# Autodesk Inventor assembly: BipeD
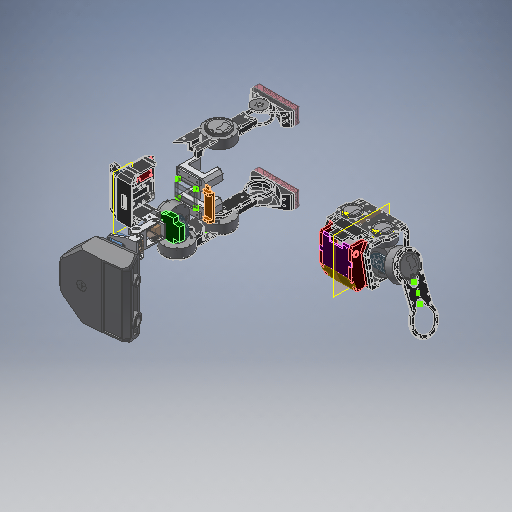
[picture p0: Inventor's stored thumbnail of the model, 512x512]
Saved by Autodesk Inventor 2026 (Build 300175000, 175)
## iProperties
Company: UNSPECIFIED
Created: 1900-01-01
Part Number: BipeD
Description: STEP AP242
Document SubType Name: Assembly
Designer: kirpe
Mass: 5721.04 g
Surface Area: 15487 cm^2
Volume: 5721.04 cm^3
Density: 1 g/cm^3
Sending System: C3D Toolkit
Preprocessor: C3D Converter
Title: Òèíêåð
Author: UNSPECIFIED
Revision Number: ANYUNSPECIFIED
## Documents named in this file (90)
- C:\BE2R\Legged_bot\biped_model\BipeD.iam
- C:\BE2R\Legged_bot\biped_model\Заднее_Ребро.ipt
- C:\BE2R\Legged_bot\biped_model\Переднее_Ребро.ipt
- C:\BE2R\Legged_bot\biped_model\Днище_Корпуса.ipt
- C:\BE2R\Legged_bot\biped_model\Булка.ipt
- C:\BE2R\Legged_bot\biped_model\Булка_1.ipt
- C:\BE2R\Legged_bot\biped_model\Держатель_ТазаV2.ipt
- C:\BE2R\Legged_bot\biped_model\DM_8006.ipt
- C:\BE2R\Legged_bot\biped_model\DM_8006_1.ipt
- C:\BE2R\Legged_bot\biped_model\Держатель_ТазаV2_1.ipt
- C:\BE2R\Legged_bot\biped_model\Тазовая_Прокладка.ipt
- C:\BE2R\Legged_bot\biped_model\БедроV2.ipt
- C:\BE2R\Legged_bot\biped_model\Голень.ipt
- C:\BE2R\Legged_bot\biped_model\Наполнитель_Бедра2.ipt
- C:\BE2R\Legged_bot\biped_model\Наполнитель Голени.ipt
- C:\BE2R\Legged_bot\biped_model\Прокладка_Стопы.ipt
- C:\BE2R\Legged_bot\biped_model\БедроV2_1.ipt
- C:\BE2R\Legged_bot\biped_model\Наполнитель_Бедра2_1.ipt
- C:\BE2R\Legged_bot\biped_model\Наполнитель Голени_1.ipt
- C:\BE2R\Legged_bot\biped_model\Голень_1.ipt
- C:\BE2R\Legged_bot\biped_model\Прокладка_Стопы_1.ipt
- C:\BE2R\Legged_bot\biped_model\НагрудникV2.ipt
- C:\BE2R\Legged_bot\biped_model\Расширитель_РюкзакаV2.ipt
- C:\BE2R\Legged_bot\biped_model\Плата.ipt
- C:\BE2R\Legged_bot\biped_model\Расширитель_РюкзакаV2_1.ipt
- C:\BE2R\Legged_bot\biped_model\СтопаV3.ipt
- C:\BE2R\Legged_bot\biped_model\СтопаV3_1.ipt
- C:\BE2R\Legged_bot\biped_model\Голова.ipt
- C:\BE2R\Legged_bot\biped_model\Шея_Верх.ipt
- C:\BE2R\Legged_bot\biped_model\Шея_Низ.ipt
- C:\BE2R\Legged_bot\biped_model\Крышка_Корпуса.ipt
- C:\BE2R\Legged_bot\biped_model\Крышка_Тумблера.ipt
- C:\BE2R\Legged_bot\biped_model\Стул.ipt
- C:\BE2R\Legged_bot\biped_model\Тумблер.ipt
- C:\BE2R\Legged_bot\biped_model\Качалка_SCS125.ipt
- C:\BE2R\Legged_bot\biped_model\Feetech_SERVO_SCS125.ipt
- C:\BE2R\Legged_bot\biped_model\FeeTech_SCS40.ipt
- C:\BE2R\Legged_bot\biped_model\Тазовая_Прокладка_1.ipt
- C:\BE2R\Legged_bot\biped_model\Кость_Таза.ipt
- C:\BE2R\Legged_bot\biped_model\Кость_Таза_1.ipt
- C:\BE2R\Legged_bot\biped_model\Кассета1.ipt
- C:\BE2R\Legged_bot\biped_model\Кассета2.ipt
- C:\BE2R\Legged_bot\biped_model\Рамка_Рюкзака.ipt
- C:\BE2R\Legged_bot\biped_model\Винт с цилиндрической головкой и шестигранным углублением под ключ ГОСТ Р ИСО 4762 -М3 x 10.ipt
- C:\BE2R\Legged_bot\biped_model\Винт с цилиндрической головкой и шестигранным углублением под ключ ГОСТ Р ИСО 4762-М3 x 6.ipt
- C:\BE2R\Legged_bot\biped_model\Винт с цилиндрической головкой и шестигранным углублением под ключ ГОСТ Р ИСО 4762-М3 x 12.ipt
- C:\BE2R\Legged_bot\biped_model\Винт с цилиндрической головкой и шестигранным углублением под ключ ГОСТ Р ИСО 4762 -М4 x 8.ipt
- C:\BE2R\Legged_bot\biped_model\Винт с цилиндрической головкой и шестигранным углублением под ключ ГОСТ Р ИСО 4762 -М3 x 16.ipt
- C:\BE2R\Legged_bot\biped_model\Винт с цилиндрической головкой и шестигранным углублением под ключ ГОСТ Р ИСО 4762 -М4 x 10.ipt
- C:\BE2R\Legged_bot\biped_model\Винт с цилиндрической головкой и шестигранным углублением под ключ ГОСТ Р ИСО 4762 -М3 x 10_1.ipt
- C:\BE2R\Legged_bot\biped_model\Винт с цилиндрической головкой и шестигранным углублением под ключ ГОСТ Р ИСО 4762-М3 x 6_1.ipt
- C:\BE2R\Legged_bot\biped_model\Винт с цилиндрической головкой и шестигранным углублением под ключ ГОСТ Р ИСО 4762-М3 x 12_1.ipt
- C:\BE2R\Legged_bot\biped_model\Винт с цилиндрической головкой и шестигранным углублением под ключ ГОСТ Р ИСО 4762 -М3 x 16_1.ipt
- C:\BE2R\Legged_bot\biped_model\Винт с цилиндрической головкой и шестигранным углублением под ключ ГОСТ Р ИСО 4762 -М4 x 10_1.ipt
- C:\BE2R\Legged_bot\biped_model\Винт с цилиндрической головкой и шестигранным углублением под ключ ГОСТ Р ИСО 4762 -М4 x 8_1.ipt
- C:\BE2R\Legged_bot\biped_model\Винт с плоской головкой ГОСТ Р ИСО 1580 -М3 x 8.ipt
- C:\BE2R\Legged_bot\biped_model\Винт с плоской головкой ГОСТ Р ИСО 1580 -М3 x 8_1.ipt
- C:\BE2R\Legged_bot\biped_model\Скамейка.ipt
- C:\BE2R\Legged_bot\biped_model\Гайка М3-6H.NF ГОСТ Р 50273-92.ipt
- C:\BE2R\Legged_bot\biped_model\Гайка М3-6H.NF ГОСТ Р 50273-92_1.ipt
- C:\BE2R\Legged_bot\biped_model\Винт с цилиндрической головкой и шестигранным углублением под ключ ГОСТ Р ИСО 4762 -М5 x 16.ipt
- C:\BE2R\Legged_bot\biped_model\Винт с цилиндрической головкой и шестигранным углублением под ключ ГОСТ Р ИСО 4762 -М5 x 16_1.ipt
- C:\BE2R\Legged_bot\biped_model\Гайка М3-6H.NF ГОСТ Р 50273-92_2.ipt
- C:\BE2R\Legged_bot\biped_model\Гайка М3-6H.NF ГОСТ Р 50273-92_3.ipt
- C:\BE2R\Legged_bot\biped_model\Винт с цилиндрической головкой и шестигранным углублением под ключ ГОСТ Р ИСО 4762 -М3 x 20.ipt
- C:\BE2R\Legged_bot\biped_model\Винт с цилиндрической головкой и шестигранным углублением под ключ ГОСТ Р ИСО 4762 -М4 x 20.ipt
- C:\BE2R\Legged_bot\biped_model\Гайка М4-6H.NF ГОСТ Р 50273-92.ipt
- C:\BE2R\Legged_bot\biped_model\Винт с цилиндрической головкой и шестигранным углублением под ключ ГОСТ Р ИСО 4762 -М4 x 12.ipt
- C:\BE2R\Legged_bot\biped_model\Винт с цилиндрической головкой и шестигранным углублением под ключ ГОСТ Р ИСО 4762 -М4 x 16.ipt
- C:\BE2R\Legged_bot\biped_model\Винт с цилиндрической головкой и шестигранным углублением под ключ ГОСТ Р ИСО 4762 -М3 x 20_1.ipt
- C:\BE2R\Legged_bot\biped_model\Винт с плоской головкой ГОСТ Р ИСО 1580 -М3 x 6.ipt
- C:\BE2R\Legged_bot\biped_model\Винт с цилиндрической головкой и шестигранным углублением под ключ ГОСТ Р ИСО 4762 -М3 x 5.ipt
- C:\BE2R\Legged_bot\biped_model\Винт с цилиндрической головкой и шестигранным углублением под ключ ГОСТ Р ИСО 4762-М2,5 x 12.ipt
- C:\BE2R\Legged_bot\biped_model\Гайка М2,5-6H ГОСТ 5916-70.ipt
- C:\BE2R\Legged_bot\biped_model\Тинкер.ipt
- C:\BE2R\Legged_bot\biped_model\Крышка_Платы_Питания.ipt
- C:\BE2R\Legged_bot\biped_model\Переднее_Ребро_1.ipt
- C:\BE2R\Legged_bot\biped_model\Нагрудник_Сторона.ipt
- C:\BE2R\Legged_bot\biped_model\Нагрудник_Сторона_1.ipt
- C:\BE2R\Legged_bot\biped_model\Нагрудник_Низ.ipt
- C:\BE2R\Legged_bot\biped_model\Нагрудник_Середина.ipt
- C:\BE2R\Legged_bot\biped_model\Нагрудник_Центр.ipt
- C:\BE2R\Legged_bot\biped_model\Рюкзак.ipt
- C:\BE2R\Legged_bot\biped_model\Крышка_Рюкзака.ipt
- C:\BE2R\Legged_bot\biped_model\Подставка_Платы.ipt
- C:\BE2R\Legged_bot\biped_model\NONE.ipt
- C:\BE2R\Legged_bot\biped_model\Башмак.ipt
- C:\BE2R\Legged_bot\biped_model\Башмак_1.ipt
- C:\BE2R\Legged_bot\biped_model\Датчик.ipt
- C:\BE2R\Legged_bot\biped_model\DM-J6006.ipt
## Components (355 placed, 86 different names)
1. Заднее_Ребро — Совмещение:10, Совмещение:11, Совмещение:12, Совмещение:41, Совмещение:42
2. Заднее_Ребро:1 — Совмещение:1, Совмещение:2, Совмещение:3, Совмещение:43
3. Переднее_Ребро — Совмещение:4, Совмещение:5, Совмещение:6, Совмещение:13, Совмещение:14, Заподлицо:1, Совмещение:15, Совмещение:16, Совмещение:17, Симметрия:1
4. Днище_Корпуса — Совмещение:13, Совмещение:14, Заподлицо:1
5. Булка
6. Булка_1
7. Держатель_ТазаV2 — Совмещение:35, Совмещение:36, Совмещение:37, Совмещение:38, Совмещение:39, Совмещение:40
8. DM_8006 — Совмещение:38, Совмещение:39, Совмещение:40, Совмещение:44, С поворотом:1
9. DM_8006_1
10. Держатель_ТазаV2_1
11. DM_8006:1 — Совмещение:48, Цилиндрический:1, Совмещение:49, Совмещение:50, Совмещение:51
12. Тазовая_Прокладка — Совмещение:45, Совмещение:46, Совмещение:47, Совмещение:48, Цилиндрический:1
13. БедроV2 — Совмещение:49, Совмещение:50, Совмещение:51
14. DM_8006:2
15. Голень
16. Наполнитель_Бедра2
17. Наполнитель Голени
18. Прокладка_Стопы
19. DM_8006_1:1
20. БедроV2_1
21. Наполнитель_Бедра2_1
22. DM_8006_1:2
23. Наполнитель Голени_1
24. Голень_1
25. Прокладка_Стопы_1
26. НагрудникV2
27. Расширитель_РюкзакаV2
28. Плата
29. Расширитель_РюкзакаV2_1
30. СтопаV3
31. СтопаV3_1
32. Голова
33. Шея_Верх
34. Шея_Низ
35. Крышка_Корпуса — Совмещение:1, Совмещение:2, Совмещение:3, Совмещение:4, Совмещение:5, Совмещение:6, Совмещение:7, Совмещение:8, Совмещение:9, Совмещение:10, Совмещение:11, Совмещение:12, Совмещение:26, Совмещение:27, Совмещение:28, Совмещение:29, Совмещение:30, Совмещение:31, Совмещение:32, Совмещение:33, Совмещение:34
36. Крышка_Тумблера — Совмещение:26, Совмещение:27, Совмещение:28
37. Стул
38. Тумблер
39. Качалка_SCS125
40. Feetech_SERVO_SCS125
41. Качалка_SCS125:1
42. FeeTech_SCS40
43. FeeTech_SCS40:1
44. Качалка_SCS125:2
45. Тазовая_Прокладка_1
46. Кость_Таза — Совмещение:44, С поворотом:1, Совмещение:45, Совмещение:46, Совмещение:47
47. Кость_Таза_1
48. Кассета1
49. Кассета2
50. Рамка_Рюкзака
51. Ключ
52. Крышка_Платы_Питания
53. Переднее_Ребро_1 — Совмещение:7, Совмещение:8, Совмещение:9, Совмещение:18, Совмещение:19, Совмещение:20, Симметрия:1
54. Нагрудник_Сторона — Совмещение:18, Совмещение:19, Совмещение:20, Заподлицо:2, Совмещение:23, Совмещение:24
55. Нагрудник_Сторона_1 — Совмещение:15, Совмещение:16, Совмещение:17, Совмещение:21, Совмещение:22, Совмещение:25
56. Нагрудник_Низ
57. Нагрудник_Середина — Совмещение:23, Совмещение:24, Совмещение:25
58. Нагрудник_Центр — Совмещение:21, Заподлицо:2, Совмещение:22
59. Рюкзак
60. -01
61. Подставка_Платы — Совмещение:41, Совмещение:42, Совмещение:43
62. Плата_Es_To CAN
63. Башмак
64. Башмак_1
65. Датчик
66. DM-J6006:1 — Совмещение:32, Совмещение:33, Совмещение:34
67. DM-J6006:2 — Совмещение:29, Совмещение:30, Совмещение:31, Совмещение:35, Совмещение:36, Совмещение:37
68. Винт с цилиндрической головкой и шестигранным углублением под ключ ГОСТ Р ИСО 4762 -М3 x 10:1
69. Винт с цилиндрической головкой и шестигранным углублением под ключ ГОСТ Р ИСО 4762 -М3 x 10:2
70. Винт с цилиндрической головкой и шестигранным углублением под ключ ГОСТ Р ИСО 4762 -М3 x 10:3
71. Винт с цилиндрической головкой и шестигранным углублением под ключ ГОСТ Р ИСО 4762 -М3 x 10:4
72. Винт с цилиндрической головкой и шестигранным углублением под ключ ГОСТ Р ИСО 4762 -М3 x 10:5
73. Винт с цилиндрической головкой и шестигранным углублением под ключ ГОСТ Р ИСО 4762-М3 x 6
74. Винт с цилиндрической головкой и шестигранным углублением под ключ ГОСТ Р ИСО 4762-М3 x 6:1
75. Винт с цилиндрической головкой и шестигранным углублением под ключ ГОСТ Р ИСО 4762-М3 x 6:2
76. Винт с цилиндрической головкой и шестигранным углублением под ключ ГОСТ Р ИСО 4762-М3 x 6:3
77. Винт с цилиндрической головкой и шестигранным углублением под ключ ГОСТ Р ИСО 4762-М3 x 6:4
78. Винт с цилиндрической головкой и шестигранным углублением под ключ ГОСТ Р ИСО 4762-М3 x 12
79. Винт с цилиндрической головкой и шестигранным углублением под ключ ГОСТ Р ИСО 4762-М3 x 12:1
80. Винт с цилиндрической головкой и шестигранным углублением под ключ ГОСТ Р ИСО 4762-М3 x 12:2
81. Винт с цилиндрической головкой и шестигранным углублением под ключ ГОСТ Р ИСО 4762-М3 x 12:3
82. Винт с цилиндрической головкой и шестигранным углублением под ключ ГОСТ Р ИСО 4762 -М4 x 8
83. Винт с цилиндрической головкой и шестигранным углублением под ключ ГОСТ Р ИСО 4762 -М4 x 8:1
84. Винт с цилиндрической головкой и шестигранным углублением под ключ ГОСТ Р ИСО 4762 -М4 x 8:2
85. Винт с цилиндрической головкой и шестигранным углублением под ключ ГОСТ Р ИСО 4762 -М4 x 8:3
86. Винт с цилиндрической головкой и шестигранным углублением под ключ ГОСТ Р ИСО 4762 -М4 x 8:4
87. Винт с цилиндрической головкой и шестигранным углублением под ключ ГОСТ Р ИСО 4762 -М4 x 8:5
88. Винт с цилиндрической головкой и шестигранным углублением под ключ ГОСТ Р ИСО 4762 -М4 x 8:6
89. Винт с цилиндрической головкой и шестигранным углублением под ключ ГОСТ Р ИСО 4762 -М4 x 8:7
90. Винт с цилиндрической головкой и шестигранным углублением под ключ ГОСТ Р ИСО 4762 -М4 x 8:8
91. Винт с цилиндрической головкой и шестигранным углублением под ключ ГОСТ Р ИСО 4762 -М4 x 8:9
92. Винт с цилиндрической головкой и шестигранным углублением под ключ ГОСТ Р ИСО 4762 -М4 x 8:10
93. Винт с цилиндрической головкой и шестигранным углублением под ключ ГОСТ Р ИСО 4762 -М4 x 8:11
94. Винт с цилиндрической головкой и шестигранным углублением под ключ ГОСТ Р ИСО 4762 -М4 x 8:12
95. Винт с цилиндрической головкой и шестигранным углублением под ключ ГОСТ Р ИСО 4762 -М3 x 10:6
96. Винт с цилиндрической головкой и шестигранным углублением под ключ ГОСТ Р ИСО 4762 -М3 x 10:7
97. Винт с цилиндрической головкой и шестигранным углублением под ключ ГОСТ Р ИСО 4762 -М3 x 16
98. Винт с цилиндрической головкой и шестигранным углублением под ключ ГОСТ Р ИСО 4762 -М3 x 16:1
99. Винт с цилиндрической головкой и шестигранным углублением под ключ ГОСТ Р ИСО 4762 -М3 x 16:2
100. Винт с цилиндрической головкой и шестигранным углублением под ключ ГОСТ Р ИСО 4762 -М3 x 16:3
101. Винт с цилиндрической головкой и шестигранным углублением под ключ ГОСТ Р ИСО 4762 -М4 x 8:13
102. Винт с цилиндрической головкой и шестигранным углублением под ключ ГОСТ Р ИСО 4762 -М4 x 8:14
103. Винт с цилиндрической головкой и шестигранным углублением под ключ ГОСТ Р ИСО 4762 -М4 x 8:15
104. Винт с цилиндрической головкой и шестигранным углублением под ключ ГОСТ Р ИСО 4762 -М4 x 8:16
105. Винт с цилиндрической головкой и шестигранным углублением под ключ ГОСТ Р ИСО 4762 -М4 x 8:17
106. Винт с цилиндрической головкой и шестигранным углублением под ключ ГОСТ Р ИСО 4762 -М4 x 8:18
107. Винт с цилиндрической головкой и шестигранным углублением под ключ ГОСТ Р ИСО 4762 -М4 x 8:19
108. Винт с цилиндрической головкой и шестигранным углублением под ключ ГОСТ Р ИСО 4762 -М4 x 10
109. Винт с цилиндрической головкой и шестигранным углублением под ключ ГОСТ Р ИСО 4762 -М4 x 10:1
110. Винт с цилиндрической головкой и шестигранным углублением под ключ ГОСТ Р ИСО 4762 -М4 x 10:2
111. Винт с цилиндрической головкой и шестигранным углублением под ключ ГОСТ Р ИСО 4762 -М4 x 10:3
112. Винт с цилиндрической головкой и шестигранным углублением под ключ ГОСТ Р ИСО 4762 -М3 x 10_1
113. Винт с цилиндрической головкой и шестигранным углублением под ключ ГОСТ Р ИСО 4762 -М3 x 10_1:1
114. Винт с цилиндрической головкой и шестигранным углублением под ключ ГОСТ Р ИСО 4762-М3 x 6_1
115. Винт с цилиндрической головкой и шестигранным углублением под ключ ГОСТ Р ИСО 4762-М3 x 6_1:1
116. Винт с цилиндрической головкой и шестигранным углублением под ключ ГОСТ Р ИСО 4762-М3 x 6_1:2
117. Винт с цилиндрической головкой и шестигранным углублением под ключ ГОСТ Р ИСО 4762-М3 x 6_1:3
118. Винт с цилиндрической головкой и шестигранным углублением под ключ ГОСТ Р ИСО 4762-М3 x 6_1:4
119. Винт с цилиндрической головкой и шестигранным углублением под ключ ГОСТ Р ИСО 4762-М3 x 12_1
120. Винт с цилиндрической головкой и шестигранным углублением под ключ ГОСТ Р ИСО 4762-М3 x 12_1:1
121. Винт с цилиндрической головкой и шестигранным углублением под ключ ГОСТ Р ИСО 4762-М3 x 12_1:2
122. Винт с цилиндрической головкой и шестигранным углублением под ключ ГОСТ Р ИСО 4762-М3 x 12_1:3
123. Винт с цилиндрической головкой и шестигранным углублением под ключ ГОСТ Р ИСО 4762 -М3 x 16_1
124. Винт с цилиндрической головкой и шестигранным углублением под ключ ГОСТ Р ИСО 4762 -М3 x 16_1:1
125. Винт с цилиндрической головкой и шестигранным углублением под ключ ГОСТ Р ИСО 4762 -М3 x 16_1:2
126. Винт с цилиндрической головкой и шестигранным углублением под ключ ГОСТ Р ИСО 4762 -М3 x 16_1:3
127. Винт с цилиндрической головкой и шестигранным углублением под ключ ГОСТ Р ИСО 4762 -М4 x 10_1
128. Винт с цилиндрической головкой и шестигранным углублением под ключ ГОСТ Р ИСО 4762 -М4 x 10_1:1
129. Винт с цилиндрической головкой и шестигранным углублением под ключ ГОСТ Р ИСО 4762 -М4 x 10_1:2
130. Винт с цилиндрической головкой и шестигранным углублением под ключ ГОСТ Р ИСО 4762 -М4 x 10_1:3
131. Винт с цилиндрической головкой и шестигранным углублением под ключ ГОСТ Р ИСО 4762 -М3 x 10_1:2
132. Винт с цилиндрической головкой и шестигранным углублением под ключ ГОСТ Р ИСО 4762 -М3 x 10_1:3
133. Винт с цилиндрической головкой и шестигранным углублением под ключ ГОСТ Р ИСО 4762 -М3 x 10_1:4
134. Винт с цилиндрической головкой и шестигранным углублением под ключ ГОСТ Р ИСО 4762 -М3 x 10_1:5
135. Винт с цилиндрической головкой и шестигранным углублением под ключ ГОСТ Р ИСО 4762 -М3 x 10_1:6
136. Винт с цилиндрической головкой и шестигранным углублением под ключ ГОСТ Р ИСО 4762 -М3 x 10_1:7
137. Винт с цилиндрической головкой и шестигранным углублением под ключ ГОСТ Р ИСО 4762 -М4 x 8_1
138. Винт с цилиндрической головкой и шестигранным углублением под ключ ГОСТ Р ИСО 4762 -М4 x 8_1:1
139. Винт с цилиндрической головкой и шестигранным углублением под ключ ГОСТ Р ИСО 4762 -М4 x 8_1:2
140. Винт с цилиндрической головкой и шестигранным углублением под ключ ГОСТ Р ИСО 4762 -М4 x 8_1:3
141. Винт с цилиндрической головкой и шестигранным углублением под ключ ГОСТ Р ИСО 4762 -М4 x 8_1:4
142. Винт с цилиндрической головкой и шестигранным углублением под ключ ГОСТ Р ИСО 4762 -М4 x 8_1:5
143. Винт с цилиндрической головкой и шестигранным углублением под ключ ГОСТ Р ИСО 4762 -М4 x 8_1:6
144. Винт с цилиндрической головкой и шестигранным углублением под ключ ГОСТ Р ИСО 4762 -М4 x 8_1:7
145. Винт с цилиндрической головкой и шестигранным углублением под ключ ГОСТ Р ИСО 4762 -М4 x 8_1:8
146. Винт с цилиндрической головкой и шестигранным углублением под ключ ГОСТ Р ИСО 4762 -М4 x 8_1:9
147. Винт с цилиндрической головкой и шестигранным углублением под ключ ГОСТ Р ИСО 4762 -М4 x 8_1:10
148. Винт с цилиндрической головкой и шестигранным углублением под ключ ГОСТ Р ИСО 4762 -М4 x 8_1:11
149. Винт с цилиндрической головкой и шестигранным углублением под ключ ГОСТ Р ИСО 4762 -М4 x 8_1:12
150. Винт с цилиндрической головкой и шестигранным углублением под ключ ГОСТ Р ИСО 4762 -М4 x 8_1:13
151. Винт с цилиндрической головкой и шестигранным углублением под ключ ГОСТ Р ИСО 4762 -М4 x 8:20
152. Винт с цилиндрической головкой и шестигранным углублением под ключ ГОСТ Р ИСО 4762 -М4 x 8:21
153. Винт с цилиндрической головкой и шестигранным углублением под ключ ГОСТ Р ИСО 4762 -М4 x 8:22
154. Винт с цилиндрической головкой и шестигранным углублением под ключ ГОСТ Р ИСО 4762 -М4 x 8:23
155. Винт с цилиндрической головкой и шестигранным углублением под ключ ГОСТ Р ИСО 4762 -М4 x 8:24
156. Винт с цилиндрической головкой и шестигранным углублением под ключ ГОСТ Р ИСО 4762 -М4 x 10:4
157. Винт с цилиндрической головкой и шестигранным углублением под ключ ГОСТ Р ИСО 4762 -М4 x 10:5
158. Винт с цилиндрической головкой и шестигранным углублением под ключ ГОСТ Р ИСО 4762 -М4 x 10:6
159. Винт с цилиндрической головкой и шестигранным углублением под ключ ГОСТ Р ИСО 4762 -М4 x 10:7
160. Винт с цилиндрической головкой и шестигранным углублением под ключ ГОСТ Р ИСО 4762 -М4 x 10:8
161. Винт с цилиндрической головкой и шестигранным углублением под ключ ГОСТ Р ИСО 4762 -М4 x 10:9
162. Винт с цилиндрической головкой и шестигранным углублением под ключ ГОСТ Р ИСО 4762-М3 x 6:5
163. Винт с цилиндрической головкой и шестигранным углублением под ключ ГОСТ Р ИСО 4762-М3 x 6:6
164. Винт с цилиндрической головкой и шестигранным углублением под ключ ГОСТ Р ИСО 4762-М3 x 6:7
165. Винт с цилиндрической головкой и шестигранным углублением под ключ ГОСТ Р ИСО 4762-М3 x 6:8
166. Винт с цилиндрической головкой и шестигранным углублением под ключ ГОСТ Р ИСО 4762-М3 x 6:9
167. Винт с плоской головкой ГОСТ Р ИСО 1580 -М3 x 8
168. Винт с плоской головкой ГОСТ Р ИСО 1580 -М3 x 8:1
169. Винт с плоской головкой ГОСТ Р ИСО 1580 -М3 x 8:2
170. Винт с плоской головкой ГОСТ Р ИСО 1580 -М3 x 8:3
171. Винт с плоской головкой ГОСТ Р ИСО 1580 -М3 x 8:4
172. Винт с плоской головкой ГОСТ Р ИСО 1580 -М3 x 8:5
173. Винт с цилиндрической головкой и шестигранным углублением под ключ ГОСТ Р ИСО 4762 -М4 x 10_1:4
174. Винт с цилиндрической головкой и шестигранным углублением под ключ ГОСТ Р ИСО 4762 -М4 x 10_1:5
175. Винт с цилиндрической головкой и шестигранным углублением под ключ ГОСТ Р ИСО 4762 -М4 x 10_1:6
176. Винт с цилиндрической головкой и шестигранным углублением под ключ ГОСТ Р ИСО 4762 -М4 x 10_1:7
177. Винт с цилиндрической головкой и шестигранным углублением под ключ ГОСТ Р ИСО 4762 -М4 x 10_1:8
178. Винт с цилиндрической головкой и шестигранным углублением под ключ ГОСТ Р ИСО 4762 -М4 x 10_1:9
179. Винт с цилиндрической головкой и шестигранным углублением под ключ ГОСТ Р ИСО 4762 -М4 x 10_1:10
180. Винт с цилиндрической головкой и шестигранным углублением под ключ ГОСТ Р ИСО 4762 -М4 x 10_1:11
181. Винт с цилиндрической головкой и шестигранным углублением под ключ ГОСТ Р ИСО 4762 -М4 x 10_1:12
182. Винт с цилиндрической головкой и шестигранным углублением под ключ ГОСТ Р ИСО 4762 -М4 x 10_1:13
183. Винт с цилиндрической головкой и шестигранным углублением под ключ ГОСТ Р ИСО 4762 -М4 x 8_1:14
184. Винт с цилиндрической головкой и шестигранным углублением под ключ ГОСТ Р ИСО 4762 -М4 x 8_1:15
185. Винт с цилиндрической головкой и шестигранным углублением под ключ ГОСТ Р ИСО 4762 -М4 x 8_1:16
186. Винт с цилиндрической головкой и шестигранным углублением под ключ ГОСТ Р ИСО 4762 -М4 x 8_1:17
187. Винт с цилиндрической головкой и шестигранным углублением под ключ ГОСТ Р ИСО 4762 -М4 x 8_1:18
188. Винт с цилиндрической головкой и шестигранным углублением под ключ ГОСТ Р ИСО 4762-М3 x 6_1:5
189. Винт с цилиндрической головкой и шестигранным углублением под ключ ГОСТ Р ИСО 4762-М3 x 6_1:6
190. Винт с цилиндрической головкой и шестигранным углублением под ключ ГОСТ Р ИСО 4762-М3 x 6_1:7
191. Винт с цилиндрической головкой и шестигранным углублением под ключ ГОСТ Р ИСО 4762-М3 x 6_1:8
192. Винт с цилиндрической головкой и шестигранным углублением под ключ ГОСТ Р ИСО 4762-М3 x 6_1:9
193. Винт с плоской головкой ГОСТ Р ИСО 1580 -М3 x 8_1
194. Винт с плоской головкой ГОСТ Р ИСО 1580 -М3 x 8_1:1
195. Винт с плоской головкой ГОСТ Р ИСО 1580 -М3 x 8_1:2
196. Винт с плоской головкой ГОСТ Р ИСО 1580 -М3 x 8_1:3
197. Винт с плоской головкой ГОСТ Р ИСО 1580 -М3 x 8_1:4
198. Винт с плоской головкой ГОСТ Р ИСО 1580 -М3 x 8_1:5
199. Скамейка
200. Скамейка:1
201. Гайка М3-6H
202. Гайка М3-6H:1
203. Гайка М3-6H:2
204. Гайка М3-6H:3
205. Гайка М3-6H:4
206. Гайка М3-6H:5
207. Гайка М3-6H:6
208. Гайка М3-6H:7
209. Гайка М3-6H:8
210. Гайка М3-6H:9
211. Гайка М3-6H:10
212. Гайка М3-6H:11
213. Винт с цилиндрической головкой и шестигранным углублением под ключ ГОСТ Р ИСО 4762 -М4 x 8_1:19
214. Винт с цилиндрической головкой и шестигранным углублением под ключ ГОСТ Р ИСО 4762 -М4 x 8_1:20
215. Винт с цилиндрической головкой и шестигранным углублением под ключ ГОСТ Р ИСО 4762 -М4 x 8_1:21
216. Винт с цилиндрической головкой и шестигранным углублением под ключ ГОСТ Р ИСО 4762 -М4 x 8_1:22
217. Винт с цилиндрической головкой и шестигранным углублением под ключ ГОСТ Р ИСО 4762 -М4 x 8_1:23
218. Винт с цилиндрической головкой и шестигранным углублением под ключ ГОСТ Р ИСО 4762 -М4 x 8_1:24
219. Гайка М3-6H:12
220. Гайка М3-6H:13
221. Гайка М3-6H:14
222. Гайка М3-6H:15
223. Винт с цилиндрической головкой и шестигранным углублением под ключ ГОСТ Р ИСО 4762 -М5 x 16
224. Винт с цилиндрической головкой и шестигранным углублением под ключ ГОСТ Р ИСО 4762 -М5 x 16:1
225. Гайка М3-6H:16
226. Гайка М3-6H:17
227. Гайка М3-6H:18
228. Гайка М3-6H:19
229. Винт с цилиндрической головкой и шестигранным углублением под ключ ГОСТ Р ИСО 4762 -М3 x 16:4
230. Винт с цилиндрической головкой и шестигранным углублением под ключ ГОСТ Р ИСО 4762 -М3 x 16:5
231. Винт с цилиндрической головкой и шестигранным углублением под ключ ГОСТ Р ИСО 4762 -М3 x 16:6
232. Винт с цилиндрической головкой и шестигранным углублением под ключ ГОСТ Р ИСО 4762 -М3 x 16:7
233. Гайка М3-6H:20
234. Винт с цилиндрической головкой и шестигранным углублением под ключ ГОСТ Р ИСО 4762 -М3 x 16_1:4
235. Винт с цилиндрической головкой и шестигранным углублением под ключ ГОСТ Р ИСО 4762 -М3 x 16_1:5
236. Гайка М3-6H:21
237. Винт с цилиндрической головкой и шестигранным углублением под ключ ГОСТ Р ИСО 4762 -М3 x 16_1:6
238. Гайка М3-6H:22
239. Гайка М3-6H:23
240. Винт с цилиндрической головкой и шестигранным углублением под ключ ГОСТ Р ИСО 4762 -М3 x 16_1:7
241. Винт с цилиндрической головкой и шестигранным углублением под ключ ГОСТ Р ИСО 4762 -М5 x 16_1
242. Винт с цилиндрической головкой и шестигранным углублением под ключ ГОСТ Р ИСО 4762 -М5 x 16_1:1
243. Винт с цилиндрической головкой и шестигранным углублением под ключ ГОСТ Р ИСО 4762-М3 x 12:4
244. Винт с цилиндрической головкой и шестигранным углублением под ключ ГОСТ Р ИСО 4762-М3 x 12:5
245. Винт с цилиндрической головкой и шестигранным углублением под ключ ГОСТ Р ИСО 4762-М3 x 12:6
246. Винт с цилиндрической головкой и шестигранным углублением под ключ ГОСТ Р ИСО 4762-М3 x 12:7
247. Винт с цилиндрической головкой и шестигранным углублением под ключ ГОСТ Р ИСО 4762-М3 x 12:8
248. Винт с цилиндрической головкой и шестигранным углублением под ключ ГОСТ Р ИСО 4762-М3 x 12:9
249. Винт с цилиндрической головкой и шестигранным углублением под ключ ГОСТ Р ИСО 4762-М3 x 12:10
250. Винт с цилиндрической головкой и шестигранным углублением под ключ ГОСТ Р ИСО 4762-М3 x 12:11
251. Винт с цилиндрической головкой и шестигранным углублением под ключ ГОСТ Р ИСО 4762-М3 x 12:12
252. Винт с цилиндрической головкой и шестигранным углублением под ключ ГОСТ Р ИСО 4762-М3 x 12:13
253. Винт с цилиндрической головкой и шестигранным углублением под ключ ГОСТ Р ИСО 4762-М3 x 12:14
254. Винт с цилиндрической головкой и шестигранным углублением под ключ ГОСТ Р ИСО 4762-М3 x 12:15
255. Гайка М3-6H:24
256. Гайка М3-6H:25
257. Винт с цилиндрической головкой и шестигранным углублением под ключ ГОСТ Р ИСО 4762-М3 x 12_1:4
258. Гайка М3-6H:26
259. Винт с цилиндрической головкой и шестигранным углублением под ключ ГОСТ Р ИСО 4762-М3 x 12_1:5
260. Винт с цилиндрической головкой и шестигранным углублением под ключ ГОСТ Р ИСО 4762-М3 x 12_1:6
261. Винт с цилиндрической головкой и шестигранным углублением под ключ ГОСТ Р ИСО 4762-М3 x 12_1:7
262. Гайка М3-6H:27
263. Винт с цилиндрической головкой и шестигранным углублением под ключ ГОСТ Р ИСО 4762-М3 x 12_1:8
264. Винт с цилиндрической головкой и шестигранным углублением под ключ ГОСТ Р ИСО 4762-М3 x 12_1:9
265. Винт с цилиндрической головкой и шестигранным углублением под ключ ГОСТ Р ИСО 4762-М3 x 12_1:10
266. Винт с цилиндрической головкой и шестигранным углублением под ключ ГОСТ Р ИСО 4762-М3 x 12_1:11
267. Винт с цилиндрической головкой и шестигранным углублением под ключ ГОСТ Р ИСО 4762-М3 x 12_1:12
268. Винт с цилиндрической головкой и шестигранным углублением под ключ ГОСТ Р ИСО 4762-М3 x 12_1:13
269. Винт с цилиндрической головкой и шестигранным углублением под ключ ГОСТ Р ИСО 4762-М3 x 12_1:14
270. Винт с цилиндрической головкой и шестигранным углублением под ключ ГОСТ Р ИСО 4762-М3 x 12_1:15
271. Гайка М3-6H:28
272. Винт с цилиндрической головкой и шестигранным углублением под ключ ГОСТ Р ИСО 4762 -М3 x 20
273. Винт с цилиндрической головкой и шестигранным углублением под ключ ГОСТ Р ИСО 4762 -М4 x 20
274. Гайка М4-6H
275. Гайка М4-6H:1
276. Гайка М4-6H:2
277. Гайка М4-6H:3
278. Гайка М4-6H:4
279. Гайка М4-6H:5
280. Гайка М4-6H:6
281. Гайка М4-6H:7
282. Гайка М4-6H:8
283. Гайка М4-6H:9
284. Гайка М4-6H:10
285. Винт с цилиндрической головкой и шестигранным углублением под ключ ГОСТ Р ИСО 4762 -М4 x 12
286. Винт с цилиндрической головкой и шестигранным углублением под ключ ГОСТ Р ИСО 4762 -М4 x 12:1
287. Винт с цилиндрической головкой и шестигранным углублением под ключ ГОСТ Р ИСО 4762 -М4 x 12:2
288. Винт с цилиндрической головкой и шестигранным углублением под ключ ГОСТ Р ИСО 4762 -М4 x 12:3
289. Винт с цилиндрической головкой и шестигранным углублением под ключ ГОСТ Р ИСО 4762 -М4 x 16
290. Винт с цилиндрической головкой и шестигранным углублением под ключ ГОСТ Р ИСО 4762 -М4 x 16:1
291. Винт с цилиндрической головкой и шестигранным углублением под ключ ГОСТ Р ИСО 4762 -М4 x 16:2
292. Винт с цилиндрической головкой и шестигранным углублением под ключ ГОСТ Р ИСО 4762 -М4 x 16:3
293. Винт с цилиндрической головкой и шестигранным углублением под ключ ГОСТ Р ИСО 4762 -М4 x 20:1
294. Винт с цилиндрической головкой и шестигранным углублением под ключ ГОСТ Р ИСО 4762 -М4 x 20:2
295. Винт с цилиндрической головкой и шестигранным углублением под ключ ГОСТ Р ИСО 4762 -М3 x 20_1
296. Гайка М3-6H:29
297. Винт с цилиндрической головкой и шестигранным углублением под ключ ГОСТ Р ИСО 4762 -М4 x 20:3
298. Гайка М4-6H:11
299. Винт с плоской головкой ГОСТ Р ИСО 1580 -М3 x 8:6
300. Винт с плоской головкой ГОСТ Р ИСО 1580 -М3 x 8:7
301. Винт с плоской головкой ГОСТ Р ИСО 1580 -М3 x 8:8
302. Винт с плоской головкой ГОСТ Р ИСО 1580 -М3 x 8:9
303. Винт с плоской головкой ГОСТ Р ИСО 1580 -М3 x 8:10
304. Винт с плоской головкой ГОСТ Р ИСО 1580 -М3 x 8:11
305. Винт с плоской головкой ГОСТ Р ИСО 1580 -М3 x 8:12
306. Винт с плоской головкой ГОСТ Р ИСО 1580 -М3 x 8:13
307. Винт с плоской головкой ГОСТ Р ИСО 1580 -М3 x 8:14
308. Винт с плоской головкой ГОСТ Р ИСО 1580 -М3 x 8:15
309. Винт с плоской головкой ГОСТ Р ИСО 1580 -М3 x 8:16
310. Винт с плоской головкой ГОСТ Р ИСО 1580 -М3 x 8:17
311. Винт с плоской головкой ГОСТ Р ИСО 1580 -М3 x 6
312. Винт с плоской головкой ГОСТ Р ИСО 1580 -М3 x 6:1
313. Винт с плоской головкой ГОСТ Р ИСО 1580 -М3 x 6:2
314. Винт с плоской головкой ГОСТ Р ИСО 1580 -М3 x 6:3
315. Винт с плоской головкой ГОСТ Р ИСО 1580 -М3 x 6:4
316. Винт с плоской головкой ГОСТ Р ИСО 1580 -М3 x 6:5
317. Винт с плоской головкой ГОСТ Р ИСО 1580 -М3 x 6:6
318. Винт с плоской головкой ГОСТ Р ИСО 1580 -М3 x 6:7
319. Винт с цилиндрической головкой и шестигранным углублением под ключ ГОСТ Р ИСО 4762 -М3 x 5
320. Винт с цилиндрической головкой и шестигранным углублением под ключ ГОСТ Р ИСО 4762 -М3 x 5:1
321. Винт с цилиндрической головкой и шестигранным углублением под ключ ГОСТ Р ИСО 4762 -М3 x 5:2
322. Винт с цилиндрической головкой и шестигранным углублением под ключ ГОСТ Р ИСО 4762 -М3 x 5:3
323. Винт с цилиндрической головкой и шестигранным углублением под ключ ГОСТ Р ИСО 4762-М2,5 x 12
324. Гайка М2,5-6H ГОСТ 5916-70
325. Гайка М2,5-6H ГОСТ 5916-70:1
326. Гайка М2,5-6H ГОСТ 5916-70:2
327. Гайка М2,5-6H ГОСТ 5916-70:3
328. Гайка М2,5-6H ГОСТ 5916-70:4
329. Гайка М2,5-6H ГОСТ 5916-70:5
330. Гайка М2,5-6H ГОСТ 5916-70:6
331. Гайка М2,5-6H ГОСТ 5916-70:7
332. Гайка М2,5-6H ГОСТ 5916-70:8
333. Гайка М2,5-6H ГОСТ 5916-70:9
334. Гайка М2,5-6H ГОСТ 5916-70:10
335. Гайка М2,5-6H ГОСТ 5916-70:11
336. Винт с цилиндрической головкой и шестигранным углублением под ключ ГОСТ Р ИСО 4762-М2,5 x 12:1
337. Винт с цилиндрической головкой и шестигранным углублением под ключ ГОСТ Р ИСО 4762-М2,5 x 12:2
338. Винт с цилиндрической головкой и шестигранным углублением под ключ ГОСТ Р ИСО 4762-М2,5 x 12:3
339. Винт с цилиндрической головкой и шестигранным углублением под ключ ГОСТ Р ИСО 4762-М2,5 x 12:4
340. Винт с цилиндрической головкой и шестигранным углублением под ключ ГОСТ Р ИСО 4762-М2,5 x 12:5
341. Винт с цилиндрической головкой и шестигранным углублением под ключ ГОСТ Р ИСО 4762-М2,5 x 12:6
342. Винт с цилиндрической головкой и шестигранным углублением под ключ ГОСТ Р ИСО 4762-М2,5 x 12:7
343. Винт с цилиндрической головкой и шестигранным углублением под ключ ГОСТ Р ИСО 4762-М2,5 x 12:8
344. Винт с цилиндрической головкой и шестигранным углублением под ключ ГОСТ Р ИСО 4762-М2,5 x 12:9
345. Винт с цилиндрической головкой и шестигранным углублением под ключ ГОСТ Р ИСО 4762-М2,5 x 12:10
346. Винт с цилиндрической головкой и шестигранным углублением под ключ ГОСТ Р ИСО 4762-М2,5 x 12:11
347. Винт с цилиндрической головкой и шестигранным углублением под ключ ГОСТ Р ИСО 4762-М2,5 x 12:12
348. Винт с цилиндрической головкой и шестигранным углублением под ключ ГОСТ Р ИСО 4762-М2,5 x 12:13
349. Винт с цилиндрической головкой и шестигранным углублением под ключ ГОСТ Р ИСО 4762-М2,5 x 12:14
350. Винт с цилиндрической головкой и шестигранным углублением под ключ ГОСТ Р ИСО 4762-М2,5 x 12:15
351. Гайка М2,5-6H ГОСТ 5916-70:12
352. Гайка М2,5-6H ГОСТ 5916-70:13
353. Гайка М2,5-6H ГОСТ 5916-70:14
354. Гайка М2,5-6H ГОСТ 5916-70:15
355. Винт с цилиндрической головкой и шестигранным углублением под ключ ГОСТ Р ИСО 4762 -М3 x 10
## Relationships (56: Mate 51, Flush 2, Symmetry 1, RevoluteJoint 1, CylindricalJoint 1)
- Совмещение:1 [Mate]: Заднее_Ребро:1 ↔ Крышка_Корпуса
- Совмещение:2 [Mate]: Заднее_Ребро:1 ↔ Крышка_Корпуса
- Совмещение:3 [Mate]: Заднее_Ребро:1 ↔ Крышка_Корпуса
- Совмещение:4 [Mate]: Переднее_Ребро ↔ Крышка_Корпуса
- Совмещение:5 [Mate]: Переднее_Ребро ↔ Крышка_Корпуса
- Совмещение:6 [Mate]: Переднее_Ребро ↔ Крышка_Корпуса
- Совмещение:7 [Mate]: Крышка_Корпуса ↔ Переднее_Ребро_1
- Совмещение:8 [Mate]: Крышка_Корпуса ↔ Переднее_Ребро_1
- Совмещение:9 [Mate]: Крышка_Корпуса ↔ Переднее_Ребро_1
- Совмещение:10 [Mate]: Заднее_Ребро ↔ Крышка_Корпуса
- Совмещение:11 [Mate]: Заднее_Ребро ↔ Крышка_Корпуса
- Совмещение:12 [Mate]: Заднее_Ребро ↔ Крышка_Корпуса
- Совмещение:13 [Mate]: Переднее_Ребро ↔ Днище_Корпуса
- Совмещение:14 [Mate]: Переднее_Ребро ↔ Днище_Корпуса
- Заподлицо:1 [Flush]: Переднее_Ребро ↔ Днище_Корпуса
- Совмещение:15 [Mate]: Переднее_Ребро ↔ Нагрудник_Сторона_1
- Совмещение:16 [Mate]: Переднее_Ребро ↔ Нагрудник_Сторона_1
- Совмещение:17 [Mate]: Переднее_Ребро ↔ Нагрудник_Сторона_1
- Совмещение:18 [Mate]: Переднее_Ребро_1 ↔ Нагрудник_Сторона
- Совмещение:19 [Mate]: Переднее_Ребро_1 ↔ Нагрудник_Сторона
- Совмещение:20 [Mate]: Переднее_Ребро_1 ↔ Нагрудник_Сторона
- Совмещение:21 [Mate]: Нагрудник_Сторона_1 ↔ Нагрудник_Центр
- Заподлицо:2 [Flush]: Нагрудник_Сторона ↔ Нагрудник_Центр
- Совмещение:22 [Mate]: Нагрудник_Сторона_1 ↔ Нагрудник_Центр
- Совмещение:23 [Mate]: Нагрудник_Сторона ↔ Нагрудник_Середина
- Совмещение:24 [Mate]: Нагрудник_Сторона ↔ Нагрудник_Середина
- Совмещение:25 [Mate]: Нагрудник_Сторона_1 ↔ Нагрудник_Середина
- Симметрия:1 [Symmetry]: Переднее_Ребро ↔ Переднее_Ребро_1
- Совмещение:26 [Mate]: Крышка_Корпуса ↔ Крышка_Тумблера
- Совмещение:27 [Mate]: Крышка_Корпуса ↔ Крышка_Тумблера
- Совмещение:28 [Mate]: Крышка_Корпуса ↔ Крышка_Тумблера
- Совмещение:29 [Mate]: Крышка_Корпуса ↔ DM-J6006:2
- Совмещение:30 [Mate]: Крышка_Корпуса ↔ DM-J6006:2
- Совмещение:31 [Mate]: Крышка_Корпуса ↔ DM-J6006:2
- Совмещение:32 [Mate]: Крышка_Корпуса ↔ DM-J6006:1
- Совмещение:33 [Mate]: Крышка_Корпуса ↔ DM-J6006:1
- Совмещение:34 [Mate]: Крышка_Корпуса ↔ DM-J6006:1
- Совмещение:35 [Mate]: Держатель_ТазаV2 ↔ DM-J6006:2
- Совмещение:36 [Mate]: Держатель_ТазаV2 ↔ DM-J6006:2
- Совмещение:37 [Mate]: Держатель_ТазаV2 ↔ DM-J6006:2
- Совмещение:38 [Mate]: Держатель_ТазаV2 ↔ DM_8006
- Совмещение:39 [Mate]: Держатель_ТазаV2 ↔ DM_8006
- Совмещение:40 [Mate]: Держатель_ТазаV2 ↔ DM_8006
- Совмещение:41 [Mate]: Заднее_Ребро ↔ Подставка_Платы
- Совмещение:42 [Mate]: Заднее_Ребро ↔ Подставка_Платы
- Совмещение:43 [Mate]: Заднее_Ребро:1 ↔ Подставка_Платы
- Совмещение:44 [Mate]: DM_8006 ↔ Кость_Таза
- С поворотом:1 [RevoluteJoint]: DM_8006 ↔ Кость_Таза
- Совмещение:45 [Mate]: Тазовая_Прокладка ↔ Кость_Таза
- Совмещение:46 [Mate]: Тазовая_Прокладка ↔ Кость_Таза
- Совмещение:47 [Mate]: Тазовая_Прокладка ↔ Кость_Таза
- Совмещение:48 [Mate]: DM_8006:1 ↔ Тазовая_Прокладка
- Цилиндрический:1 [CylindricalJoint]: DM_8006:1 ↔ Тазовая_Прокладка
- Совмещение:49 [Mate]: DM_8006:1 ↔ БедроV2
- Совмещение:50 [Mate]: DM_8006:1 ↔ БедроV2
- Совмещение:51 [Mate]: DM_8006:1 ↔ БедроV2
